# Autodesk Inventor assembly: Assembly
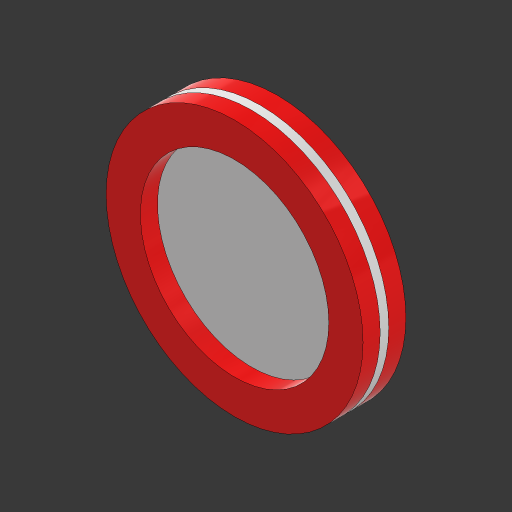
[picture p0: Inventor's stored thumbnail of the model, 512x512]
Saved by Autodesk Inventor 2023 (Build 270158000, 158)
## iProperties
Created: 2023-03-16
Part Number: Assembly
Document SubType Name: Assembly
Designer: alber
Author: alber
## Documents named in this file (3)
- C:\Users\alber\Desktop\NEARLab\dVRK\Trocar_Entry_Membrane\Assembly.iam
- C:\Users\alber\Desktop\NEARLab\dVRK\Trocar_Entry_Membrane\Membrane.ipt
- C:\Users\alber\Desktop\NEARLab\dVRK\Trocar_Entry_Membrane\Ring.ipt
## Components (3 placed, 2 different names)
1. Membrane:1 — Flush:1, Insert:1
2. Ring:1 — Flush:1
3. Ring:2 — Insert:1
## Relationships (2: Flush 1, Insert 1)
- Flush:1: Membrane:1 ↔ Ring:1
- Insert:1: Membrane:1 ↔ Ring:2
